# Autodesk Inventor assembly: dripper_assembly
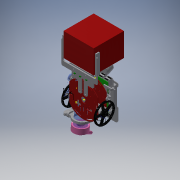
[picture p0: Inventor's stored thumbnail of the model, 180x180]
Saved by Autodesk Inventor 2017 (Build 210142000, 142)
## iProperties
Created: 2017-07-15
Part Number: dripper_assembly
Document SubType Name: Assembly
Designer: Nic
Author: Nic
## Documents named in this file (33)
- C:\Users\Nic\Documents\iDripper\dripper_assembly.iam
- C:\Users\Nic\Documents\iDripper\base_quick.ipt
- C:\Users\Nic\Documents\iDripper\motor_quick.ipt
- C:\Users\Nic\Documents\iDripper\wheel.ipt
- C:\Users\Nic\Documents\iDripper\waterbottle.ipt
- C:\Users\Nic\Documents\iDripper\tipper_link_A.ipt
- C:\Users\Nic\Documents\iDripper\tipper_link_B.ipt
- C:\Users\Nic\Documents\iDripper\waterbottle_lid.ipt
- C:\Users\Nic\Documents\iDripper\linkage_mount.ipt
- C:\Users\Nic\Documents\iDripper\RPI\RASPBERRY PI 3.ipt
- C:\Users\Nic\Documents\iDripper\tipper_link_C.ipt
- C:\Users\Nic\Documents\iDripper\tipper_link_D.ipt
- C:\Users\Nic\Documents\iDripper\waterbottle_holder_side.ipt
- C:\Users\Nic\Documents\iDripper\C01200101000M.ipt
- C:\Users\Nic\Documents\iDripper\bearing_3x4x10.ipt
- C:\Users\Nic\Documents\iDripper\nylon_shaft_7mm.ipt
- C:\Users\Nic\Documents\iDripper\nylon_shaft_13mm.ipt
- C:\Users\Nic\Documents\iDripper\washer_3x6.ipt
- C:\Users\Nic\Documents\iDripper\linkage_mount_MIR.ipt
- C:\Users\Nic\Documents\iDripper\spacer.ipt
- C:\Users\Nic\Documents\iDripper\header.ipt
- C:\Users\Nic\Documents\iDripper\shovel_mount.ipt
- C:\Users\Nic\Documents\iDripper\shovel_side.ipt
- C:\Users\Nic\Documents\iDripper\shovel.ipt
- C:\Users\Nic\Documents\iDripper\block_model.ipt
- C:\Users\Nic\Documents\iDripper\humidity_sensor.iam
- C:\Users\Nic\Documents\iDripper\humidity_support.ipt
- C:\Users\Nic\Documents\iDripper\bump_sensor_mount.ipt
- C:\Users\Nic\Documents\iDripper\shovel_support.ipt
- C:\Users\Nic\Documents\iDripper\fixed_holder.ipt
- C:\Users\Nic\Documents\iDripper\omnicam.ipt
- C:\Users\Nic\Documents\iDripper\freestanding_cam_mount.ipt
- C:\Users\Nic\Documents\iDripper\long_battery_mount.ipt
## Components (61 placed, 32 different names)
1. base_quick:1 — Slider:1, Flush:1, Slider:2, Cylindrical:1, Flush:4, Mate:17, Flush:8, Flush:9, Insert:86, Insert:87
2. base_quick:2 — Mate:1, Cylindrical:1, Flush:4, Insert:7, Insert:8, Mate:14, Mate:15, Insert:56, Insert:57, Mate:20, Insert:105
3. motor_quick:1 — Slider:1, Flush:1, Insert:1, Mate:1
4. motor_quick:2 — Slider:2, Insert:2, Mate:20, Flush:9
5. wheel:1 — Insert:1, Rotation:1
6. wheel:2 — Insert:2, Insert:35, Insert:53, Rotation:1
7. linkage_mount:1 — Insert:7, Insert:8, Insert:29, Insert:36, Insert:44, Insert:45
8. RASPBERRY PI 3:1 — Mate:18, Flush:8, Insert:82, Insert:83
9. C01200101000M:1
10. spacer:1 — Insert:83, Insert:84
11. spacer:2 — Insert:82, Insert:85
12. header:1 — Insert:84, Insert:85, Insert:97, Insert:98, Insert:111, Insert:112, Insert:113, Insert:114
13. shovel_mount:1 — Insert:86, Insert:87, Insert:88, Insert:89, Insert:101, Insert:102
14. header:2 — Insert:97, Insert:98
15. bump_sensor_mount:1 — Insert:105
16. fixed_holder:1 — Mate:30, Insert:110, Mate:32
17. omnicam:1 — Mate:39
18. shovel_support:2 — Mate:36, Flush:11, Mate:37
19. freestanding_cam_mount:1 — Insert:111, Insert:112, Mate:39
20. long_battery_mount:1 — Insert:113, Insert:114
21. tipper_link_A:1 — Insert:23, Insert:25
22. tipper_link_B:1 — Insert:27, Insert:32, Insert:42, Insert:52
23. waterbottle:2 — Insert:6
24. waterbottle_lid:1 — Insert:6, Insert:110
25. tipper_link_D:1 — Insert:30, Insert:39
26. tipper_link_C:1 — Insert:106, Insert:107, Insert:108, Insert:109, Mate:30, Mate:32
27. waterbottle_holder_side:1
28. waterbottle_holder_side:2
29. linkage_mount_MIR:1 — Insert:54, Insert:55, Insert:56, Insert:57, Insert:59, Insert:60, Mate:18
30. nylon_shaft_7mm:4 — Insert:55
31. nylon_shaft_7mm:5 — Insert:54
32. washer_3x6:7 — Insert:59
33. washer_3x6:8 — Insert:60
34. bearing_3x4x10:1 — Insert:23, Insert:46
35. bearing_3x4x10:2 — Insert:25, Insert:43
36. nylon_shaft_7mm:1 — Insert:27
37. nylon_shaft_7mm:2 — Insert:29
38. bearing_3x4x10:3 — Insert:30, Insert:37
39. bearing_3x4x10:4 — Insert:32, Insert:81
40. nylon_shaft_13mm:1 — Insert:35
41. washer_3x6:1 — Insert:36, Insert:37
42. nylon_shaft_13mm:2 — Insert:106
43. bearing_3x4x10:5 — Insert:39, Insert:41
44. washer_3x6:2 — Insert:41, Insert:48
45. washer_3x6:3 — Insert:42, Insert:43
46. nylon_shaft_7mm:3 — Insert:44
47. washer_3x6:4 — Insert:45, Insert:46
48. washer_3x6:5 — Insert:48, Insert:107
49. washer_3x6:6 — Insert:81, Insert:109
50. nylon_shaft_13mm:3 — Insert:108
51. bearing_3x4x10:6 — Insert:52, Insert:53
52. shovel_support:1 — Mate:34, Flush:10, Mate:35, Mate:38
53. shovel_side:1 — Insert:88, Insert:89, Insert:90, Insert:91
54. shovel:1 — Insert:99, Insert:100, Mate:34, Flush:10, Mate:35, Mate:36, Flush:11, Mate:37, Flush:12
55. shovel_side:2 — Insert:90, Insert:91, Insert:99, Insert:100
56. block_model:1 — Flush:12, Mate:38
57. humidity_support:1 — Insert:101, Insert:102, Insert:103, Insert:104
58. humidity_support:2 — Insert:103, Insert:104, Mate:23, Angle:2, Mate:24, Mate:25, Mate:26, Mate:27
59. humidity_sensor:1 [sub-assembly] — Mate:23, Angle:2
60. humidity_sensor:2 [sub-assembly] — Mate:24, Mate:26
61. humidity_sensor:3 [sub-assembly] — Mate:25, Mate:27
## Relationships (91: Insert 59, Mate 20, Flush 7, TranslationJoint 2, CylindricalJoint 1, RelateRotation 1, Angle 1)
- Slider:1 [TranslationJoint]: base_quick:1 ↔ motor_quick:1
- Flush:1: base_quick:1 ↔ motor_quick:1
- Slider:2 [TranslationJoint]: base_quick:1 ↔ motor_quick:2
- Mate:1: base_quick:2 ↔ motor_quick:1
- Cylindrical:1: base_quick:1 ↔ base_quick:2
- Insert:1: motor_quick:1 ↔ wheel:1
- Insert:2: motor_quick:2 ↔ wheel:2
- Insert:6: waterbottle:2 ↔ waterbottle_lid:1
- Flush:4: base_quick:1 ↔ base_quick:2
- Insert:7: base_quick:2 ↔ linkage_mount:1
- Insert:8: base_quick:2 ↔ linkage_mount:1
- Insert:23: tipper_link_A:1 ↔ bearing_3x4x10:1
- Insert:25: tipper_link_A:1 ↔ bearing_3x4x10:2
- Insert:27: tipper_link_B:1 ↔ nylon_shaft_7mm:1
- Insert:29: linkage_mount:1 ↔ nylon_shaft_7mm:2
- Insert:30: tipper_link_D:1 ↔ bearing_3x4x10:3
- Insert:32: tipper_link_B:1 ↔ bearing_3x4x10:4
- Insert:35: wheel:2 ↔ nylon_shaft_13mm:1
- Insert:36: linkage_mount:1 ↔ washer_3x6:1
- Insert:37: bearing_3x4x10:3 ↔ washer_3x6:1
- Insert:39: tipper_link_D:1 ↔ bearing_3x4x10:5
- Insert:41: bearing_3x4x10:5 ↔ washer_3x6:2
- Insert:42: tipper_link_B:1 ↔ washer_3x6:3
- Insert:43: bearing_3x4x10:2 ↔ washer_3x6:3
- Insert:44: linkage_mount:1 ↔ nylon_shaft_7mm:3
- Insert:45: linkage_mount:1 ↔ washer_3x6:4
- Insert:46: bearing_3x4x10:1 ↔ washer_3x6:4
- Insert:48: washer_3x6:2 ↔ washer_3x6:5
- Insert:52: tipper_link_B:1 ↔ bearing_3x4x10:6
- Insert:53 (8.775 mm): wheel:2 ↔ bearing_3x4x10:6
- Mate:14: base_quick:2
- Mate:15: base_quick:2
- Mate:16
- Mate:17: base_quick:1
- Insert:54: linkage_mount_MIR:1 ↔ nylon_shaft_7mm:5
- Insert:55: linkage_mount_MIR:1 ↔ nylon_shaft_7mm:4
- Insert:56: base_quick:2 ↔ linkage_mount_MIR:1
- Insert:57: base_quick:2 ↔ linkage_mount_MIR:1
- Insert:59: linkage_mount_MIR:1 ↔ washer_3x6:7
- Insert:60: linkage_mount_MIR:1 ↔ washer_3x6:8
- Mate:18: RASPBERRY PI 3:1 ↔ linkage_mount_MIR:1
- Flush:8 (-0.75 mm): base_quick:1 ↔ RASPBERRY PI 3:1
- Rotation:1 [RelateRotation] (1 ul): wheel:1 ↔ wheel:2
- Insert:81: bearing_3x4x10:4 ↔ washer_3x6:6
- Insert:82: RASPBERRY PI 3:1 ↔ spacer:2
- Insert:83: RASPBERRY PI 3:1 ↔ spacer:1
- Insert:84: spacer:1 ↔ header:1
- Insert:85: spacer:2 ↔ header:1
- Mate:20: base_quick:2 ↔ motor_quick:2
- Flush:9: base_quick:1 ↔ motor_quick:2
- Insert:86: base_quick:1 ↔ shovel_mount:1
- Insert:87: base_quick:1 ↔ shovel_mount:1
- Insert:88: shovel_mount:1 ↔ shovel_side:1
- Insert:89: shovel_mount:1 ↔ shovel_side:1
- Insert:90: shovel_side:1 ↔ shovel_side:2
- Insert:91: shovel_side:1 ↔ shovel_side:2
- Insert:97: header:1 ↔ header:2
- Insert:98: header:1 ↔ header:2
- Insert:99: shovel:1 ↔ shovel_side:2
- Insert:100: shovel:1 ↔ shovel_side:2
- Insert:101: shovel_mount:1 ↔ humidity_support:1
- Insert:102: shovel_mount:1 ↔ humidity_support:1
- Insert:103: humidity_support:1 ↔ humidity_support:2
- Insert:104: humidity_support:1 ↔ humidity_support:2
- Mate:23 (2 mm): humidity_support:2 ↔ humidity_sensor:1
- Angle:2 (0 deg): humidity_support:2 ↔ humidity_sensor:1
- Mate:24 (2 mm): humidity_support:2 ↔ humidity_sensor:2
- Mate:25 (2 mm): humidity_support:2 ↔ humidity_sensor:3
- Mate:26: humidity_support:2 ↔ humidity_sensor:2
- Mate:27: humidity_support:2 ↔ humidity_sensor:3
- Insert:105: base_quick:2 ↔ bump_sensor_mount:1
- Insert:106 (0.5 mm): tipper_link_C:1 ↔ nylon_shaft_13mm:2
- Insert:107: tipper_link_C:1 ↔ washer_3x6:5
- Insert:108: tipper_link_C:1 ↔ nylon_shaft_13mm:3
- Insert:109: tipper_link_C:1 ↔ washer_3x6:6
- Mate:30 (1 mm): fixed_holder:1 ↔ tipper_link_C:1
- Insert:110 (12 mm): fixed_holder:1 ↔ waterbottle_lid:1
- Mate:32: fixed_holder:1 ↔ tipper_link_C:1
- Mate:34: shovel_support:1 ↔ shovel:1
- Flush:10: shovel_support:1 ↔ shovel:1
- Mate:35: shovel_support:1 ↔ shovel:1
- Mate:36: shovel_support:2 ↔ shovel:1
- Flush:11: shovel_support:2 ↔ shovel:1
- Mate:37: shovel_support:2 ↔ shovel:1
- Flush:12: shovel:1 ↔ block_model:1
- Mate:38: shovel_support:1 ↔ block_model:1
- Insert:111: header:1 ↔ freestanding_cam_mount:1
- Insert:112: header:1 ↔ freestanding_cam_mount:1
- Mate:39: omnicam:1 ↔ freestanding_cam_mount:1
- Insert:113: header:1 ↔ long_battery_mount:1
- Insert:114: header:1 ↔ long_battery_mount:1
